# Autodesk Inventor assembly: 조립품1
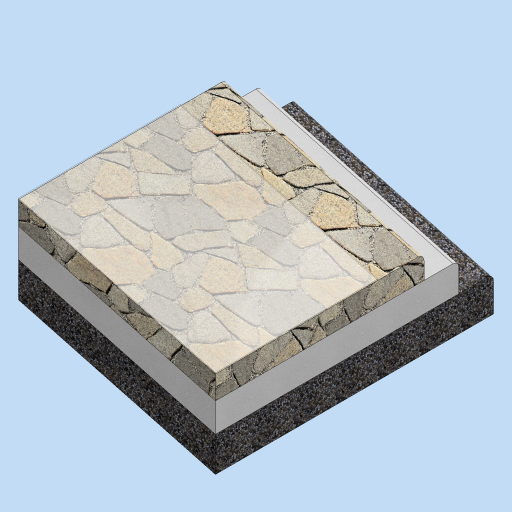
[picture p0: Inventor's stored thumbnail of the model, 512x512]
Saved by Autodesk Inventor 2024.1 (Build 281209000, 209)
## iProperties
Created: 2024-01-18
Part Number: 조립품1
Document SubType Name: Assembly
Designer: likek
Author: likek
## Documents named in this file (4)
- C:\Users\likek\Videos\Modeling\두원칼라콘크리트\[조립]5번 작업물.iam
- C:\Users\likek\Videos\Modeling\두원칼라콘크리트\5번 작업물.ipt
- C:\Users\likek\OneDrive\바탕 화면\부품3.ipt
- C:\Users\likek\Videos\Modeling\두원칼라콘크리트\코팅면.ipt
## Components (3 placed, 3 different names)
1. 5번 작업물:1 — 강체:2, 강체:3
2. 부품3:1 — 강체:2
3. 코팅면:1 — 강체:3
## Relationships (2: WeldJoint 2)
- 강체:2 [WeldJoint]: 5번 작업물:1 ↔ 부품3:1
- 강체:3 [WeldJoint]: 5번 작업물:1 ↔ 코팅면:1
